# Autodesk Inventor assembly: Phone Holder Assembly
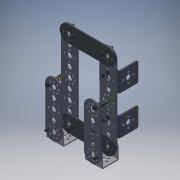
[picture p0: Inventor's stored thumbnail of the model, 180x180]
Saved by Autodesk Inventor 2016 (Build 200138000, 138)
## iProperties
Created: 2015-09-08
Part Number: Phone Holder Assembly
Document SubType Name: Assembly
Designer: phiro
Author: phiro
## Documents named in this file (10)
- C:\Users\phiro\Documents\GitHub\phi_robotics\3d-models\FTC_Tetrix_KOP_Block_Party\Tim Bloot Designs\Tutorial Bot\Phone Holder Assembly.iam
- C:\Users\phiro\Documents\GitHub\phi_robotics\3d-models\FTC_Tetrix_KOP_Block_Party\Tetrix_Kit_FTC\Autodesk Inventor Files\tetrix_739061_2012.ipt
- C:\Users\phiro\Documents\GitHub\phi_robotics\3d-models\FTC_Tetrix_KOP_Block_Party\Tetrix_Kit_FTC\Autodesk Inventor Files\tetrix_739272_2013.ipt
- C:\Users\phiro\Documents\GitHub\phi_robotics\3d-models\FTC_Tetrix_KOP_Block_Party\Tetrix_Kit_FTC\Autodesk Inventor Files\tetrix_screw-buttonhead.ipt
- C:\Users\phiro\Documents\GitHub\phi_robotics\3d-models\FTC_Tetrix_KOP_Block_Party\Tetrix_Kit_FTC\Autodesk Inventor Files\tetrix_c_channel-round.ipt
- C:\Users\phiro\Documents\GitHub\phi_robotics\3d-models\FTC_Tetrix_KOP_Block_Party\Tetrix_Kit_FTC\Autodesk Inventor Files\tetrix_inside_corner_bracket.ipt
- C:\Users\phiro\Documents\GitHub\phi_robotics\3d-models\FTC_Tetrix_KOP_Block_Party\Tetrix_Kit_FTC\Autodesk Inventor Files\tetrix_standoff_post-1in.ipt
- C:\Users\phiro\Documents\GitHub\phi_robotics\3d-models\FTC_Tetrix_KOP_Block_Party\Tetrix_Kit_FTC\Autodesk Inventor Files\tetrix_screw.ipt
- C:\Users\phiro\Documents\GitHub\phi_robotics\3d-models\FTC_Tetrix_KOP_Block_Party\Tetrix_Kit_FTC\Autodesk Inventor Files\tetrix_739273_2013.ipt
- C:\Users\phiro\Documents\GitHub\phi_robotics\3d-models\FTC_Tetrix_KOP_Block_Party\Tetrix_Kit_FTC\Autodesk Inventor Files\tetrix_screw-short.ipt
## Components (30 placed, 9 different names)
1. tetrix_739061_2012:1 — Rigid:1, Rigid:2, Rotational:1, Rotational:2, Rotational:3, Rotational:4
2. tetrix_739061_2012:2 — Rigid:5, Rigid:6, Rotational:5, Rotational:6, Rotational:7, Rotational:8
3. tetrix_739272_2013:1 — Rigid:1, Rigid:4, Rigid:5, Rigid:10, Rotational:14
4. tetrix_739272_2013:2 — Rigid:2, Rigid:3, Rigid:6, Rigid:7, Rigid:8, Rotational:9, Rotational:10, Rotational:11, Rotational:12, Rigid:9, Rotational:13
5. tetrix_screw-buttonhead:1 — Rotational:3
6. tetrix_screw-buttonhead:2 — Rotational:4
7. tetrix_screw-buttonhead:3 — Rotational:1
8. tetrix_screw-buttonhead:4 — Rotational:2
9. tetrix_c_channel-round:1 — Rigid:3, Rigid:11, Rotational:15
10. tetrix_c_channel-round:2 — Rigid:4, Rigid:12, Rotational:16
11. tetrix_screw-buttonhead:5 — Rotational:8
12. tetrix_screw-buttonhead:6 — Rotational:7
13. tetrix_screw-buttonhead:7 — Rotational:5
14. tetrix_screw-buttonhead:8 — Rotational:6
15. tetrix_inside_corner_bracket:1 — Rigid:7
16. tetrix_inside_corner_bracket:2 — Rigid:8
17. tetrix_screw-buttonhead:9 — Rotational:12
18. tetrix_screw-buttonhead:10 — Rotational:11
19. tetrix_screw-buttonhead:11 — Rotational:9
20. tetrix_screw-buttonhead:12 — Rotational:10
21. tetrix_standoff_post-1in:1 — Rigid:9
22. tetrix_standoff_post-1in:2 — Rigid:10
23. tetrix_screw:1 — Rotational:14
24. tetrix_screw:2 — Rotational:13
25. tetrix_739273_2013:1 — Rigid:12, Rotational:17
26. tetrix_739273_2013:2 — Rigid:11, Rotational:18
27. tetrix_screw-short:1 — Rotational:17
28. tetrix_screw-short:2 — Rotational:18
29. tetrix_screw-buttonhead:13 — Rotational:16
30. tetrix_screw-buttonhead:14 — Rotational:15
## Relationships (30: RevoluteJoint 18, WeldJoint 12)
- Rigid:1 [WeldJoint]: tetrix_739061_2012:1 ↔ tetrix_739272_2013:1
- Rigid:2 [WeldJoint]: tetrix_739061_2012:1 ↔ tetrix_739272_2013:2
- Rotational:1 [RevoluteJoint]: tetrix_739061_2012:1 ↔ tetrix_screw-buttonhead:3
- Rotational:2 [RevoluteJoint]: tetrix_739061_2012:1 ↔ tetrix_screw-buttonhead:4
- Rotational:3 [RevoluteJoint]: tetrix_739061_2012:1 ↔ tetrix_screw-buttonhead:1
- Rotational:4 [RevoluteJoint]: tetrix_739061_2012:1 ↔ tetrix_screw-buttonhead:2
- Rigid:3 [WeldJoint]: tetrix_739272_2013:2 ↔ tetrix_c_channel-round:1
- Rigid:4 [WeldJoint]: tetrix_739272_2013:1 ↔ tetrix_c_channel-round:2
- Rigid:5 [WeldJoint]: tetrix_739061_2012:2 ↔ tetrix_739272_2013:1
- Rigid:6 [WeldJoint]: tetrix_739061_2012:2 ↔ tetrix_739272_2013:2
- Rotational:5 [RevoluteJoint]: tetrix_739061_2012:2 ↔ tetrix_screw-buttonhead:7
- Rotational:6 [RevoluteJoint]: tetrix_739061_2012:2 ↔ tetrix_screw-buttonhead:8
- Rotational:7 [RevoluteJoint]: tetrix_739061_2012:2 ↔ tetrix_screw-buttonhead:6
- Rotational:8 [RevoluteJoint]: tetrix_739061_2012:2 ↔ tetrix_screw-buttonhead:5
- Rigid:7 [WeldJoint]: tetrix_739272_2013:2 ↔ tetrix_inside_corner_bracket:1
- Rigid:8 [WeldJoint]: tetrix_739272_2013:2 ↔ tetrix_inside_corner_bracket:2
- Rotational:9 [RevoluteJoint]: tetrix_739272_2013:2 ↔ tetrix_screw-buttonhead:11
- Rotational:10 [RevoluteJoint]: tetrix_739272_2013:2 ↔ tetrix_screw-buttonhead:12
- Rotational:11 [RevoluteJoint]: tetrix_739272_2013:2 ↔ tetrix_screw-buttonhead:10
- Rotational:12 [RevoluteJoint]: tetrix_739272_2013:2 ↔ tetrix_screw-buttonhead:9
- Rigid:9 [WeldJoint]: tetrix_739272_2013:2 ↔ tetrix_standoff_post-1in:1
- Rigid:10 [WeldJoint]: tetrix_739272_2013:1 ↔ tetrix_standoff_post-1in:2
- Rotational:13 [RevoluteJoint]: tetrix_739272_2013:2 ↔ tetrix_screw:2
- Rotational:14 [RevoluteJoint]: tetrix_739272_2013:1 ↔ tetrix_screw:1
- Rigid:11 [WeldJoint]: tetrix_c_channel-round:1 ↔ tetrix_739273_2013:2
- Rigid:12 [WeldJoint]: tetrix_c_channel-round:2 ↔ tetrix_739273_2013:1
- Rotational:15 [RevoluteJoint]: tetrix_c_channel-round:1 ↔ tetrix_screw-buttonhead:14
- Rotational:16 [RevoluteJoint]: tetrix_c_channel-round:2 ↔ tetrix_screw-buttonhead:13
- Rotational:17 [RevoluteJoint]: tetrix_739273_2013:1 ↔ tetrix_screw-short:1
- Rotational:18 [RevoluteJoint]: tetrix_739273_2013:2 ↔ tetrix_screw-short:2
